# Autodesk Inventor assembly: thumper-bumper-assm
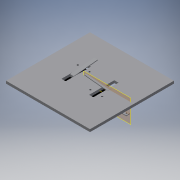
[picture p0: Inventor's stored thumbnail of the model, 180x180]
Saved by Autodesk Inventor 2017 (Build 210142000, 142)
## iProperties
Created: 2017-02-22
Part Number: thumper-bumper-assm
Document SubType Name: Assembly
Designer: John
Author: John
## Documents named in this file (3)
- C:\Users\John\Dropbox\ECE115\pinball-project\thumper-bumper-assm.iam
- C:\Users\John\Dropbox\ECE115\pinball-project\thumper-bumper-base.ipt
- C:\Users\John\Dropbox\ECE115\pinball-project\game-switch.ipt
## Components (3 placed, 2 different names)
1. thumper-bumper-base:1 — Mate:2, Mate:3, Mate:4
2. game-switch:1 — Mate:3, Mate:4
3. game-switch:2 — Mate:2
## Relationships (3: Mate 3)
- Mate:2: thumper-bumper-base:1 ↔ game-switch:2
- Mate:3: thumper-bumper-base:1 ↔ game-switch:1
- Mate:4: thumper-bumper-base:1 ↔ game-switch:1
